# Autodesk Inventor assembly: seperatorSheet
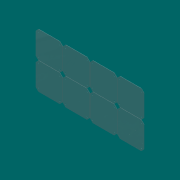
[picture p0: Inventor's stored thumbnail of the model, 180x180]
Saved by Autodesk Inventor 2016 (Build 200138000, 138)
## iProperties
Created: 2016-09-30
Part Number: seperatorSheet
Document SubType Name: Assembly
Designer: sawaiz
Author: sawaiz
## Documents named in this file (3)
- C:\Users\sawaiz\oneDrive\projects\muonTelescope\frame\separator\seperatorSheet.iam
- C:\Users\sawaiz\oneDrive\projects\muonTelescope\frame\separator\separatingPanels.ipt
- C:\Users\sawaiz\oneDrive\projects\muonTelescope\frame\separator\piMount.ipt
## Components (8 placed, 2 different names)
1. separatingPanels:1 — Flush:1, Flush:2, Flush:12, Mate:1, Mate:2
2. separatingPanels:2 — Flush:1, Flush:2, Flush:7, Flush:8, Flush:13, Mate:2, Mate:3
3. separatingPanels:3 — Flush:5, Flush:6, Flush:8, Flush:9, Flush:14, Mate:3, Mate:4
4. separatingPanels:4 — Flush:6, Flush:7, Flush:10, Flush:14, Flush:15, Flush:16
5. separatingPanels:5 — Flush:3, Flush:11, Flush:12, Mate:1
6. separatingPanels:6 — Flush:3, Flush:4, Flush:10, Flush:11, Flush:13
7. separatingPanels:7 — Flush:4, Flush:5, Flush:9, Flush:17, Mate:4
8. piMount:1 — Flush:15, Flush:16, Flush:17
## Relationships (21: Flush 17, Mate 4)
- Flush:1: separatingPanels:1 ↔ separatingPanels:2
- Flush:2: separatingPanels:1 ↔ separatingPanels:2
- Flush:3: separatingPanels:5 ↔ separatingPanels:6
- Flush:4: separatingPanels:6 ↔ separatingPanels:7
- Flush:5: separatingPanels:3 ↔ separatingPanels:7
- Flush:6: separatingPanels:3 ↔ separatingPanels:4
- Flush:7: separatingPanels:2 ↔ separatingPanels:4
- Flush:8: separatingPanels:2 ↔ separatingPanels:3
- Flush:9: separatingPanels:3 ↔ separatingPanels:7
- Flush:10: separatingPanels:4 ↔ separatingPanels:6
- Flush:11: separatingPanels:5 ↔ separatingPanels:6
- Flush:12: separatingPanels:1 ↔ separatingPanels:5
- Flush:13: separatingPanels:2 ↔ separatingPanels:6
- Flush:14: separatingPanels:3 ↔ separatingPanels:4
- Flush:15: separatingPanels:4 ↔ piMount:1
- Flush:16: separatingPanels:4 ↔ piMount:1
- Flush:17: separatingPanels:7 ↔ piMount:1
- Mate:1 (0.5 mm): separatingPanels:1 ↔ separatingPanels:5
- Mate:2 (0.5 mm): separatingPanels:1 ↔ separatingPanels:2
- Mate:3 (0.5 mm): separatingPanels:2 ↔ separatingPanels:3
- Mate:4 (0.5 mm): separatingPanels:3 ↔ separatingPanels:7
